# Autodesk Inventor assembly: both sides of drive
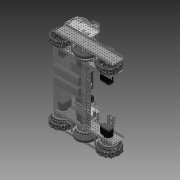
[picture p0: Inventor's stored thumbnail of the model, 180x180]
Saved by Autodesk Inventor 2014 SP1 (Build 180222100, 222)
## iProperties
Created: 2014-02-23
Part Number: both sides of drive
Document SubType Name: Assembly
Designer: Ryan
Author: Ryan
## Documents named in this file (13)
- C:\Users\Ryan\Desktop\sw\toss up 4th robot\drive\both sides of drive.iam
- C:\Users\Ryan\Desktop\sw\toss up 4th robot\drive\one side of drive.iam
- C:\Users\Ryan\Desktop\sw\lib\Aperture VEX CAD Library\Metal\L Bar\2 x 25.ipt
- C:\Users\Ryan\Desktop\sw\lib\Aperture VEX CAD Library\Metal\C Channel\5 x 25.ipt
- C:\Users\Ryan\Desktop\sw\lib\Super Sonic Sparks VEX CAD Library\Other Parts\(VEX) Cortex Microcontroller.iam
- C:\Users\Ryan\Desktop\sw\lib\Super Sonic Sparks VEX CAD Library\Other Parts\Power Expander.iam
- C:\Users\Ryan\Desktop\sw\lib\Super Sonic Sparks VEX CAD Library\Other Parts\7.2V (Robot Battery) NiMH 3000mAh.ipt
- C:\Users\Ryan\Desktop\sw\lib\Aperture VEX CAD Library\Metal\Custom 1 bar\15 mounting cortex.ipt
- C:\Users\Ryan\Desktop\sw\lib\Aperture VEX CAD Library\Spacers\SPACER-0500-0500.ipt
- C:\Users\Ryan\Desktop\sw\lib\Aperture VEX CAD Library\Spacers\SPACER-0500-0250.ipt
- C:\Users\Ryan\Desktop\sw\toss up 4th robot\drive\one side of drive_MIR.iam
- C:\Users\Ryan\Desktop\sw\toss up 4th robot\drive\pto piston.iam
- C:\Users\Ryan\Desktop\sw\toss up 4th robot\drive\battery holder poly.ipt
## Components (20 placed, 12 different names)
1. one side of drive:1 [sub-assembly] — Mate:1, Flush:1, Flush:2, Mate:2, Flush:3, Flush:4, Mate:81, Mate:83
2. 2 x 25:1 — Mate:1, Flush:1, Flush:2, Mate:16, Mate:22, Mate:80, Flush:18, Flush:19, Mate:85
3. 2 x 25:2 — Mate:2, Flush:3, Flush:4, Mate:3, Flush:5, Flush:6, Flush:12, Flush:13, Flush:14, Mate:15, Flush:15, Flush:17, Mate:66, Mate:67, Mate:68
4. 5 x 25:1 — Mate:3, Flush:5, Flush:6, Flush:20
5. 15 mounting cortex:1 — Mate:9, Flush:12, Mate:12, Flush:15, Mate:67, Mate:77, Mate:78, Mate:79
6. 15 mounting cortex:2 — Mate:10, Flush:13, Mate:11, Mate:65, Mate:66, Mate:72, Mate:73, Mate:74
7. 15 mounting cortex:3 — Flush:14, Mate:14, Flush:17, Mate:61, Mate:62, Mate:63, Mate:64, Mate:68, Mate:69
8. (VEX) Cortex Microcontroller:1 [sub-assembly] — Mate:9, Mate:10, Mate:11, Mate:12, Mate:65
9. Power Expander:1 [sub-assembly] — Mate:14, Mate:64, Mate:69
10. 7.2V (Robot Battery) NiMH 3000mAh:1 — Mate:15, Mate:16, Flush:16
11. 7.2V (Robot Battery) NiMH 3000mAh:2 — Mate:22, Flush:16
12. SPACER-0500-0500:1 — Mate:59, Mate:60, Mate:62
13. SPACER-0500-0250:1 — Mate:59, Mate:60, Mate:61, Mate:63
14. SPACER-0500-0500:2 — Mate:72, Mate:73, Mate:74
15. SPACER-0500-0250:2
16. SPACER-0500-0500:3 — Mate:77, Mate:78, Mate:79
17. SPACER-0500-0250:3
18. one side of drive_MIR:1 [sub-assembly] — Mate:80, Flush:18, Flush:19, Mate:84
19. pto piston:1 [sub-assembly] — Mate:81, Flush:21
20. battery holder poly:1 — Mate:83, Mate:84, Mate:85
## Relationships (53: Mate 37, Flush 16)
- Mate:1: one side of drive:1 ↔ 2 x 25:1
- Flush:1: one side of drive:1 ↔ 2 x 25:1
- Flush:2: one side of drive:1 ↔ 2 x 25:1
- Mate:2: one side of drive:1 ↔ 2 x 25:2
- Flush:3: one side of drive:1 ↔ 2 x 25:2
- Flush:4: one side of drive:1 ↔ 2 x 25:2
- Mate:3: 2 x 25:2 ↔ 5 x 25:1
- Flush:5: 2 x 25:2 ↔ 5 x 25:1
- Flush:6: 2 x 25:2 ↔ 5 x 25:1
- Mate:9 (2.3114 mm): 15 mounting cortex:1 ↔ (VEX) Cortex Microcontroller:1
- Mate:10 (2.3114 mm): 15 mounting cortex:2 ↔ (VEX) Cortex Microcontroller:1
- Flush:12: 2 x 25:2 ↔ 15 mounting cortex:1
- Flush:13: 2 x 25:2 ↔ 15 mounting cortex:2
- Mate:11 (2.3114 mm): 15 mounting cortex:2 ↔ (VEX) Cortex Microcontroller:1
- Mate:12 (2.3114 mm): 15 mounting cortex:1 ↔ (VEX) Cortex Microcontroller:1
- Flush:14: 2 x 25:2 ↔ 15 mounting cortex:3
- Mate:14 (2.3114 mm): 15 mounting cortex:3 ↔ Power Expander:1
- Mate:15: 2 x 25:2 ↔ 7.2V (Robot Battery) NiMH 3000mAh:1
- Mate:16: 2 x 25:1 ↔ 7.2V (Robot Battery) NiMH 3000mAh:1
- Flush:15: 2 x 25:2 ↔ 15 mounting cortex:1
- Mate:22: 2 x 25:1 ↔ 7.2V (Robot Battery) NiMH 3000mAh:2
- Flush:16: 7.2V (Robot Battery) NiMH 3000mAh:1 ↔ 7.2V (Robot Battery) NiMH 3000mAh:2
- Flush:17: 2 x 25:2 ↔ 15 mounting cortex:3
- Mate:59: SPACER-0500-0500:1 ↔ SPACER-0500-0250:1
- Mate:60: SPACER-0500-0500:1 ↔ SPACER-0500-0250:1
- Mate:61: 15 mounting cortex:3 ↔ SPACER-0500-0250:1
- Mate:62 (2.3114 mm): 15 mounting cortex:3 ↔ SPACER-0500-0500:1
- Mate:63 (2.3114 mm): 15 mounting cortex:3 ↔ SPACER-0500-0250:1
- Mate:64: 15 mounting cortex:3 ↔ Power Expander:1
- Mate:65: 15 mounting cortex:2 ↔ (VEX) Cortex Microcontroller:1
- Mate:66: 2 x 25:2 ↔ 15 mounting cortex:2
- Mate:67: 2 x 25:2 ↔ 15 mounting cortex:1
- Mate:68: 2 x 25:2 ↔ 15 mounting cortex:3
- Mate:69 (2.3114 mm): 15 mounting cortex:3 ↔ Power Expander:1
- [Mate]: SPACER-0500-0500:2 ↔ SPACER-0500-0250:2
- [Mate]: SPACER-0500-0500:2 ↔ SPACER-0500-0250:2
- Mate:72 (2.3114 mm): 15 mounting cortex:2 ↔ SPACER-0500-0500:2
- Mate:73 (2.3114 mm): 15 mounting cortex:2 ↔ SPACER-0500-0500:2
- Mate:74: 15 mounting cortex:2 ↔ SPACER-0500-0500:2
- [Mate]: SPACER-0500-0500:3 ↔ SPACER-0500-0250:3
- [Mate]: SPACER-0500-0500:3 ↔ SPACER-0500-0250:3
- Mate:77 (2.3114 mm): 15 mounting cortex:1 ↔ SPACER-0500-0500:3
- Mate:78 (2.3114 mm): 15 mounting cortex:1 ↔ SPACER-0500-0500:3
- Mate:79: 15 mounting cortex:1 ↔ SPACER-0500-0500:3
- Mate:80: 2 x 25:1 ↔ one side of drive_MIR:1
- Flush:18: 2 x 25:1 ↔ one side of drive_MIR:1
- Flush:19: 2 x 25:1 ↔ one side of drive_MIR:1
- Mate:81: one side of drive:1 ↔ pto piston:1
- Flush:20 (2.3114 mm): 5 x 25:1
- Flush:21 (-88.8619 mm): pto piston:1
- Mate:83: one side of drive:1 ↔ battery holder poly:1
- Mate:84: one side of drive_MIR:1 ↔ battery holder poly:1
- Mate:85: 2 x 25:1 ↔ battery holder poly:1
## Named parameters: q = 2.3114 mm, d91_d80 = 0 mm, d92_d81 = 0 mm, d96_d80 = 0 mm, d97_d81 = 0 mm
